# Autodesk Inventor assembly: Bot Assembly
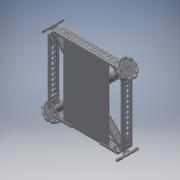
[picture p0: Inventor's stored thumbnail of the model, 180x180]
Saved by Autodesk Inventor 2019 (Build 230136000, 136)
## iProperties
Created: 2018-12-27
Part Number: Bot Assembly
Document SubType Name: Assembly
Designer: Ashley
Author: Ashley
## Documents named in this file (20)
- C:\Users\mrhftc\repositories\design\inventor\2018-2019\Body Assemblies\Bot Assembly.iam
- C:\Users\mrhftc\repositories\design\inventor\Imported Components\goBilda\Low-Side-Channel 336mm.ipt
- C:\Users\mrhftc\repositories\design\inventor\2018-2019\Body Assemblies\Wheel Corner.ipt
- C:\Users\mrhftc\repositories\design\inventor\2018-2019\Body Assemblies\Base Assembly\Design Accelerator\Bolted Connection1.iam
- C:\Users\mrhftc\repositories\design\inventor\2018-2019\Body Assemblies\Base Assembly\Design Accelerator\Bolted Connection2.iam
- C:\Users\mrhftc\repositories\design\inventor\2018-2019\Body Assemblies\Base Assembly\Design Accelerator\Bolted Connection3.iam
- C:\Users\mrhftc\repositories\design\inventor\2018-2019\Body Assemblies\Base Assembly\Design Accelerator\Bolted Connection4.iam
- C:\Users\mrhftc\repositories\design\inventor\2018-2019\Body Assemblies\Base Assembly\Design Accelerator\Bolted Connection5.iam
- C:\Users\mrhftc\repositories\design\inventor\2018-2019\Body Assemblies\Base Assembly\Design Accelerator\Bolted Connection6.iam
- C:\Users\mrhftc\repositories\design\inventor\2018-2019\Body Assemblies\Base Assembly\Design Accelerator\Bolted Connection7.iam
- C:\Users\mrhftc\repositories\design\inventor\2018-2019\Body Assemblies\Base Assembly\Design Accelerator\Bolted Connection8.iam
- C:\Users\mrhftc\repositories\design\inventor\Imported Components\goBilda\Motor\Yellow Jacket Planetary Gear Motor.ipt
- C:\Users\mrhftc\repositories\design\inventor\2018-2019\Body Assemblies\Base Assembly\Design Accelerator\Bolted Connection9.iam
- C:\Users\mrhftc\repositories\design\inventor\2018-2019\Body Assemblies\Base Assembly\Design Accelerator\Bolted Connection10.iam
- C:\Users\mrhftc\repositories\design\inventor\2018-2019\Body Assemblies\Base Assembly\Design Accelerator\Bolted Connection11.iam
- C:\Users\mrhftc\repositories\design\inventor\2018-2019\Body Assemblies\Base Assembly\Design Accelerator\Bolted Connection12.iam
- C:\Users\mrhftc\repositories\design\inventor\2018-2019\Body Assemblies\Wheels_hubs.iam
- C:\Users\mrhftc\repositories\design\inventor\Imported Components\goBilda\Thrust Bearing\Thrust Bearing.iam
- C:\Users\mrhftc\repositories\design\inventor\Imported Components\goBilda\Low-Side-U-Channel, 3 Hole, 96mm.ipt
- C:\Users\mrhftc\repositories\design\inventor\2018-2019\Body Assemblies\Base Assembly\Plexiglass Base\Plexiglass base.ipt
## Components (34 placed, 8 different names)
1. Low-Side-Channel 336mm:2 — Mate:6, Mate:7, Mate:8, Mate:9, Mate:10, Mate:11, Mate:24, Mate:25, Mate:26, Mate:27, Mate:28, Mate:29, Mate:30, Mate:31, Mate:32
2. Low-Side-Channel 336mm:3 — Mate:1, Mate:2, Mate:3, Mate:4, Mate:5, Mate:15, Mate:16, Mate:17, Mate:18, Mate:19, Mate:20, Mate:21, Mate:22, Mate:23, Mate:66, Mate:67, Mate:68, Mate:73, Mate:74, Rotational:4
3. Low-Side-Channel 336mm:4 — Mate:50, Mate:51, Mate:52, Mate:53, Mate:54, Mate:55, Mate:56, Mate:57, Mate:58, Mate:59, Mate:60, Mate:61, Mate:62, Mate:63, Mate:64, Mate:65, Mate:69, Mate:70, Rotational:3
4. Wheel Corner:1 — Mate:50, Mate:51, Mate:52, Mate:53, Mate:54, Mate:55, Mate:56, Mate:57, Mate:79, Mate:80, Mate:81, Mate:82, Mate:91, Mate:92, Rotational:2
5. Wheel Corner:2 — Mate:9, Mate:28, Mate:29, Mate:30, Mate:31, Mate:32, Mate:83, Mate:84, Mate:85, Mate:86, Mate:93, Mate:94, Rotational:1
6. Wheel Corner:3 — Mate:1, Mate:6, Mate:21, Mate:22, Mate:23, Mate:24, Mate:25, Mate:26, Mate:27, Mate:87, Mate:88, Mate:89, Mate:90, Mate:95, Mate:96
7. Wheel Corner:4 — Mate:15, Mate:16, Mate:17, Mate:18, Mate:19, Mate:20, Mate:58, Mate:59, Mate:60, Mate:61, Mate:62, Mate:63, Mate:64, Mate:65, Mate:66, Mate:67, Mate:68, Mate:75, Mate:76, Mate:77, Mate:78, Mate:97, Mate:98, Rotational:3
8. Bolted Connection:1 [sub-assembly] — Mate:2, Mate:3
9. Bolted Connection:2 [sub-assembly] — Mate:4, Mate:5
10. Bolted Connection:3 [sub-assembly] — Mate:7, Mate:8
11. Bolted Connection:4 [sub-assembly] — Mate:10, Mate:11
12. Bolted Connection:5 [sub-assembly]
13. Bolted Connection:6 [sub-assembly] — Mate:69, Mate:70
14. Bolted Connection:7 [sub-assembly]
15. Bolted Connection:8 [sub-assembly] — Mate:73, Mate:74
16. Yellow Jacket Planetary Gear Motor:1 — Mate:87, Mate:88, Mate:89, Mate:90, Insert:4, Insert:6
17. Yellow Jacket Planetary Gear Motor:2 — Mate:75, Mate:76, Mate:77, Mate:78, Insert:1, Insert:5
18. Yellow Jacket Planetary Gear Motor:3 — Mate:79, Mate:80, Mate:81, Mate:82, Insert:2, Insert:8
19. Yellow Jacket Planetary Gear Motor:4 — Mate:83, Mate:84, Mate:85, Mate:86, Insert:3, Insert:7
20. Bolted Connection:9 [sub-assembly] — Mate:91, Mate:92
21. Bolted Connection:10 [sub-assembly] — Mate:93, Mate:94
22. Bolted Connection:11 [sub-assembly] — Mate:95, Mate:96
23. Bolted Connection:12 [sub-assembly] — Mate:97, Mate:98
24. Wheels_hubs:3 [sub-assembly] — Insert:7
25. Wheels_hubs:5 [sub-assembly] — Insert:8
26. Wheels_hubs:6 [sub-assembly] — Insert:6
27. Wheels_hubs:7 [sub-assembly] — Insert:5
28. Thrust Bearing:1 [sub-assembly] — Insert:4
29. Thrust Bearing:2 [sub-assembly] — Insert:1
30. Thrust Bearing:3 [sub-assembly] — Insert:2
31. Thrust Bearing:4 [sub-assembly] — Insert:3
32. Low-Side-U-Channel, 3 Hole, 96mm:1 — Rotational:1
33. Low-Side-U-Channel, 3 Hole, 96mm:3 — Rotational:2
34. Plexiglass base:1 — Rotational:4
## Relationships (88: Mate 76, Insert 8, RevoluteJoint 4)
- Mate:1: Low-Side-Channel 336mm:3 ↔ Wheel Corner:3
- Mate:2: Low-Side-Channel 336mm:3 ↔ Bolted Connection:1
- Mate:3: Low-Side-Channel 336mm:3 ↔ Bolted Connection:1
- Mate:4: Low-Side-Channel 336mm:3 ↔ Bolted Connection:2
- Mate:5: Low-Side-Channel 336mm:3 ↔ Bolted Connection:2
- Mate:6: Low-Side-Channel 336mm:2 ↔ Wheel Corner:3
- Mate:7: Low-Side-Channel 336mm:2 ↔ Bolted Connection:3
- Mate:8: Low-Side-Channel 336mm:2 ↔ Bolted Connection:3
- Mate:9: Low-Side-Channel 336mm:2 ↔ Wheel Corner:2
- Mate:10: Low-Side-Channel 336mm:2 ↔ Bolted Connection:4
- Mate:11: Low-Side-Channel 336mm:2 ↔ Bolted Connection:4
- Mate:15: Low-Side-Channel 336mm:3 ↔ Wheel Corner:4
- Mate:16: Low-Side-Channel 336mm:3 ↔ Wheel Corner:4
- Mate:17: Low-Side-Channel 336mm:3 ↔ Wheel Corner:4
- Mate:18: Low-Side-Channel 336mm:3 ↔ Wheel Corner:4
- Mate:19: Low-Side-Channel 336mm:3 ↔ Wheel Corner:4
- Mate:20: Low-Side-Channel 336mm:3 ↔ Wheel Corner:4
- Mate:21: Low-Side-Channel 336mm:3 ↔ Wheel Corner:3
- Mate:22: Low-Side-Channel 336mm:3 ↔ Wheel Corner:3
- Mate:23: Low-Side-Channel 336mm:3 ↔ Wheel Corner:3
- Mate:24: Low-Side-Channel 336mm:2 ↔ Wheel Corner:3
- Mate:25: Low-Side-Channel 336mm:2 ↔ Wheel Corner:3
- Mate:26: Low-Side-Channel 336mm:2 ↔ Wheel Corner:3
- Mate:27: Low-Side-Channel 336mm:2 ↔ Wheel Corner:3
- Mate:28: Low-Side-Channel 336mm:2 ↔ Wheel Corner:2
- Mate:29: Low-Side-Channel 336mm:2 ↔ Wheel Corner:2
- Mate:30: Low-Side-Channel 336mm:2 ↔ Wheel Corner:2
- Mate:31: Low-Side-Channel 336mm:2 ↔ Wheel Corner:2
- Mate:32: Low-Side-Channel 336mm:2 ↔ Wheel Corner:2
- Mate:50: Low-Side-Channel 336mm:4 ↔ Wheel Corner:1
- Mate:51: Low-Side-Channel 336mm:4 ↔ Wheel Corner:1
- Mate:52: Low-Side-Channel 336mm:4 ↔ Wheel Corner:1
- Mate:53: Low-Side-Channel 336mm:4 ↔ Wheel Corner:1
- Mate:54: Low-Side-Channel 336mm:4 ↔ Wheel Corner:1
- Mate:55: Low-Side-Channel 336mm:4 ↔ Wheel Corner:1
- Mate:56: Low-Side-Channel 336mm:4 ↔ Wheel Corner:1
- Mate:57: Low-Side-Channel 336mm:4 ↔ Wheel Corner:1
- Mate:58: Low-Side-Channel 336mm:4 ↔ Wheel Corner:4
- Mate:59: Low-Side-Channel 336mm:4 ↔ Wheel Corner:4
- Mate:60: Low-Side-Channel 336mm:4 ↔ Wheel Corner:4
- Mate:61: Low-Side-Channel 336mm:4 ↔ Wheel Corner:4
- Mate:62: Low-Side-Channel 336mm:4 ↔ Wheel Corner:4
- Mate:63: Low-Side-Channel 336mm:4 ↔ Wheel Corner:4
- Mate:64: Low-Side-Channel 336mm:4 ↔ Wheel Corner:4
- Mate:65: Low-Side-Channel 336mm:4 ↔ Wheel Corner:4
- Mate:66: Low-Side-Channel 336mm:3 ↔ Wheel Corner:4
- Mate:67: Low-Side-Channel 336mm:3 ↔ Wheel Corner:4
- Mate:68: Low-Side-Channel 336mm:3 ↔ Wheel Corner:4
- Mate:69: Low-Side-Channel 336mm:4 ↔ Bolted Connection:6
- Mate:70: Low-Side-Channel 336mm:4 ↔ Bolted Connection:6
- Mate:73: Low-Side-Channel 336mm:3 ↔ Bolted Connection:8
- Mate:74: Low-Side-Channel 336mm:3 ↔ Bolted Connection:8
- Mate:75: Wheel Corner:4 ↔ Yellow Jacket Planetary Gear Motor:2
- Mate:76: Wheel Corner:4 ↔ Yellow Jacket Planetary Gear Motor:2
- Mate:77: Wheel Corner:4 ↔ Yellow Jacket Planetary Gear Motor:2
- Mate:78: Wheel Corner:4 ↔ Yellow Jacket Planetary Gear Motor:2
- Mate:79: Wheel Corner:1 ↔ Yellow Jacket Planetary Gear Motor:3
- Mate:80: Wheel Corner:1 ↔ Yellow Jacket Planetary Gear Motor:3
- Mate:81: Wheel Corner:1 ↔ Yellow Jacket Planetary Gear Motor:3
- Mate:82: Wheel Corner:1 ↔ Yellow Jacket Planetary Gear Motor:3
- Mate:83: Wheel Corner:2 ↔ Yellow Jacket Planetary Gear Motor:4
- Mate:84: Wheel Corner:2 ↔ Yellow Jacket Planetary Gear Motor:4
- Mate:85: Wheel Corner:2 ↔ Yellow Jacket Planetary Gear Motor:4
- Mate:86: Wheel Corner:2 ↔ Yellow Jacket Planetary Gear Motor:4
- Mate:87: Wheel Corner:3 ↔ Yellow Jacket Planetary Gear Motor:1
- Mate:88: Wheel Corner:3 ↔ Yellow Jacket Planetary Gear Motor:1
- Mate:89: Wheel Corner:3 ↔ Yellow Jacket Planetary Gear Motor:1
- Mate:90: Wheel Corner:3 ↔ Yellow Jacket Planetary Gear Motor:1
- Mate:91: Wheel Corner:1 ↔ Bolted Connection:9
- Mate:92: Wheel Corner:1 ↔ Bolted Connection:9
- Mate:93: Wheel Corner:2 ↔ Bolted Connection:10
- Mate:94: Wheel Corner:2 ↔ Bolted Connection:10
- Mate:95: Wheel Corner:3 ↔ Bolted Connection:11
- Mate:96: Wheel Corner:3 ↔ Bolted Connection:11
- Mate:97: Wheel Corner:4 ↔ Bolted Connection:12
- Mate:98: Wheel Corner:4 ↔ Bolted Connection:12
- Insert:1 (-18.5 mm): Yellow Jacket Planetary Gear Motor:2 ↔ Thrust Bearing:2
- Insert:2 (-18.5 mm): Yellow Jacket Planetary Gear Motor:3 ↔ Thrust Bearing:3
- Insert:3 (-18.5 mm): Yellow Jacket Planetary Gear Motor:4 ↔ Thrust Bearing:4
- Insert:4 (-18.5 mm): Yellow Jacket Planetary Gear Motor:1 ↔ Thrust Bearing:1
- Insert:5 (-13.5 mm): Yellow Jacket Planetary Gear Motor:2 ↔ Wheels_hubs:7
- Insert:6 (-13.5 mm): Yellow Jacket Planetary Gear Motor:1 ↔ Wheels_hubs:6
- Insert:7 (-13.5 mm): Yellow Jacket Planetary Gear Motor:4 ↔ Wheels_hubs:3
- Insert:8 (-13.5 mm): Yellow Jacket Planetary Gear Motor:3 ↔ Wheels_hubs:5
- Rotational:1 [RevoluteJoint]: Wheel Corner:2 ↔ Low-Side-U-Channel, 3 Hole, 96mm:1
- Rotational:2 [RevoluteJoint]: Wheel Corner:1 ↔ Low-Side-U-Channel, 3 Hole, 96mm:3
- Rotational:3 [RevoluteJoint]: Low-Side-Channel 336mm:4 ↔ Wheel Corner:4
- Rotational:4 [RevoluteJoint]: Low-Side-Channel 336mm:3 ↔ Plexiglass base:1
